# Autodesk Inventor assembly: parte móvil
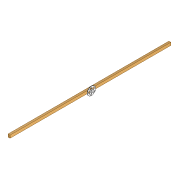
[picture p0: Inventor's stored thumbnail of the model, 180x180]
Saved by Autodesk Inventor 2020 (Build 240168000, 168)
## iProperties
Created: 2022-05-05
Part Number: parte móvil
Document SubType Name: Assembly
Designer: leo
Author: leo
## Documents named in this file (3)
- C:\Users\leo.DESKTOP-592E5E6\Documents\GitHub\TallerDix2022\cad\Inventor\parte móvil.iam
- C:\Users\leo.DESKTOP-592E5E6\Documents\GitHub\TallerDix2022\cad\Inventor\pieza.ipt
- C:\Users\leo.DESKTOP-592E5E6\Documents\GitHub\TallerDix2022\cad\Inventor\Caja\partes transmision\Polea Dentada Grande.ipt
## Components (2 placed, 2 different names)
1. pieza:1 — Insert:1
2. Polea Dentada Grande:1 — Insert:1, Flush:1
## Relationships (2: Insert 1, Flush 1)
- Insert:1 (10 mm): pieza:1 ↔ Polea Dentada Grande:1
- Flush:1: Polea Dentada Grande:1
